# Autodesk Inventor assembly: Internal Wide Panels
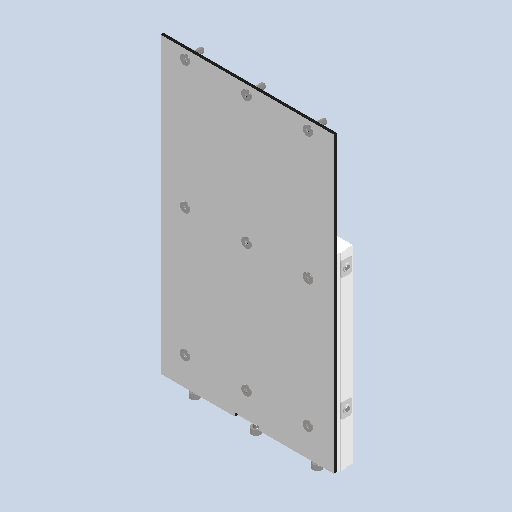
[picture p0: Inventor's stored thumbnail of the model, 512x512]
Saved by Autodesk Inventor 2024 (Build 280153000, 153)
## iProperties
Created: 2024-09-28
Part Number: Internal Wide Panels
Document SubType Name: Assembly
Designer: Ishaan
Author: Ishaan
## Documents named in this file (8)
- E:\Projects\Axiom--IDEX-3D-Printer\CAD\08 - Side Panelling\Internal Wide Panels.iam
- E:\Projects\Axiom--IDEX-3D-Printer\CAD\08 - Side Panelling\Internal medium panel supports.ipt
- E:\Projects\Axiom--IDEX-3D-Printer\CAD\08 - Side Panelling\Medium Internal Vertical Side Panels.ipt
- E:\Projects\Axiom--IDEX-3D-Printer\CAD\00 - COTS Components\Hardware\SHCSM5x12.ipt
- E:\Projects\Axiom--IDEX-3D-Printer\CAD\00 - COTS Components\Hardware\M5 LOCKNUT.ipt
- E:\Projects\Axiom--IDEX-3D-Printer\CAD\00 - COTS Components\Hardware\M5 T SLOT NUT.ipt
- E:\Projects\Axiom--IDEX-3D-Printer\CAD\00 - COTS Components\Hardware\Low Profile M5x16.ipt
- E:\Projects\Axiom--IDEX-3D-Printer\CAD\00 - COTS Components\Hardware\SHCSM5x16.ipt
## Components (31 placed, 7 different names)
1. Internal medium panel supports:1 — Insert:1, Insert:2, Insert:3, Insert:4, Insert:5, Insert:6, Insert:7, Insert:8, Insert:9, Insert:10, Insert:11, Insert:12, Insert:13, Insert:14, Insert:15, Insert:16, Insert:17, Insert:18, Insert:19, Angle:1, Angle:2, Angle:3, Angle:4, Angle:5, Angle:6, Angle:7, Angle:8, Angle:9, Insert:20, Insert:21, Insert:22, Insert:23, Angle:10, Angle:11, Angle:12, Angle:13, Insert:33, Insert:34, Insert:35
2. Medium Internal Vertical Side Panels:1 — Insert:1, Insert:2, Insert:3, Insert:4, Insert:5, Insert:6, Insert:24, Insert:25, Insert:26, Insert:27, Insert:28, Insert:29, Insert:30, Insert:31, Insert:32
3. SHCSM5x12:1 — Insert:10
4. SHCSM5x12:2 — Insert:9
5. SHCSM5x12:3 — Insert:8
6. SHCSM5x12:4 — Insert:7
7. M5 LOCKNUT:1 — Insert:17, Angle:3
8. M5 LOCKNUT:2 — Insert:15, Angle:8
9. M5 LOCKNUT:3 — Insert:18, Angle:2
10. M5 LOCKNUT:4 — Insert:19, Angle:1
11. M5 LOCKNUT:5 — Insert:16, Angle:9
12. M5 LOCKNUT:6 — Insert:14, Angle:7
13. M5 LOCKNUT:7 — Insert:11, Angle:6
14. M5 LOCKNUT:8 — Insert:12, Angle:5
15. M5 LOCKNUT:9 — Insert:13, Angle:4
16. M5 T SLOT NUT:1 — Insert:23, Angle:10
17. M5 T SLOT NUT:2 — Insert:22, Angle:11
18. M5 T SLOT NUT:3 — Insert:21, Angle:13
19. M5 T SLOT NUT:4 — Insert:20, Angle:12
20. Low Profile M5x16:1 — Insert:24
21. Low Profile M5x16:5 — Insert:32
22. Low Profile M5x16:6 — Insert:25
23. Low Profile M5x16:7 — Insert:26
24. Low Profile M5x16:8 — Insert:30
25. Low Profile M5x16:9 — Insert:31
26. Low Profile M5x16:10 — Insert:29
27. Low Profile M5x16:11 — Insert:28
28. Low Profile M5x16:12 — Insert:27
29. SHCSM5x16:1 — Insert:33
30. SHCSM5x16:2 — Insert:35
31. SHCSM5x16:3 — Insert:34
## Relationships (48: Insert 35, Angle 13)
- Insert:1: Internal medium panel supports:1 ↔ Medium Internal Vertical Side Panels:1
- Insert:2: Internal medium panel supports:1 ↔ Medium Internal Vertical Side Panels:1
- Insert:3: Internal medium panel supports:1 ↔ Medium Internal Vertical Side Panels:1
- Insert:4: Internal medium panel supports:1 ↔ Medium Internal Vertical Side Panels:1
- Insert:5: Internal medium panel supports:1 ↔ Medium Internal Vertical Side Panels:1
- Insert:6: Internal medium panel supports:1 ↔ Medium Internal Vertical Side Panels:1
- Insert:7: Internal medium panel supports:1 ↔ SHCSM5x12:4
- Insert:8: Internal medium panel supports:1 ↔ SHCSM5x12:3
- Insert:9: Internal medium panel supports:1 ↔ SHCSM5x12:2
- Insert:10: Internal medium panel supports:1 ↔ SHCSM5x12:1
- Insert:11: Internal medium panel supports:1 ↔ M5 LOCKNUT:7
- Insert:12: Internal medium panel supports:1 ↔ M5 LOCKNUT:8
- Insert:13: Internal medium panel supports:1 ↔ M5 LOCKNUT:9
- Insert:14: Internal medium panel supports:1 ↔ M5 LOCKNUT:6
- Insert:15: Internal medium panel supports:1 ↔ M5 LOCKNUT:2
- Insert:16: Internal medium panel supports:1 ↔ M5 LOCKNUT:5
- Insert:17: Internal medium panel supports:1 ↔ M5 LOCKNUT:1
- Insert:18: Internal medium panel supports:1 ↔ M5 LOCKNUT:3
- Insert:19: Internal medium panel supports:1 ↔ M5 LOCKNUT:4
- Angle:1 (0 deg): Internal medium panel supports:1 ↔ M5 LOCKNUT:4
- Angle:2 (0 deg): Internal medium panel supports:1 ↔ M5 LOCKNUT:3
- Angle:3 (0 deg): Internal medium panel supports:1 ↔ M5 LOCKNUT:1
- Angle:4 (0 deg): Internal medium panel supports:1 ↔ M5 LOCKNUT:9
- Angle:5 (0 deg): Internal medium panel supports:1 ↔ M5 LOCKNUT:8
- Angle:6 (0 deg): Internal medium panel supports:1 ↔ M5 LOCKNUT:7
- Angle:7 (0 deg): Internal medium panel supports:1 ↔ M5 LOCKNUT:6
- Angle:8 (0 deg): Internal medium panel supports:1 ↔ M5 LOCKNUT:2
- Angle:9 (0 deg): Internal medium panel supports:1 ↔ M5 LOCKNUT:5
- Insert:20 (2 mm): Internal medium panel supports:1 ↔ M5 T SLOT NUT:4
- Insert:21 (2 mm): Internal medium panel supports:1 ↔ M5 T SLOT NUT:3
- Insert:22 (2 mm): Internal medium panel supports:1 ↔ M5 T SLOT NUT:2
- Insert:23 (2 mm): Internal medium panel supports:1 ↔ M5 T SLOT NUT:1
- Angle:10 (0 deg): Internal medium panel supports:1 ↔ M5 T SLOT NUT:1
- Angle:11 (0 deg): Internal medium panel supports:1 ↔ M5 T SLOT NUT:2
- Angle:12 (0 deg): Internal medium panel supports:1 ↔ M5 T SLOT NUT:4
- Angle:13 (0 deg): Internal medium panel supports:1 ↔ M5 T SLOT NUT:3
- Insert:24: Medium Internal Vertical Side Panels:1 ↔ Low Profile M5x16:1
- Insert:25: Medium Internal Vertical Side Panels:1 ↔ Low Profile M5x16:6
- Insert:26: Medium Internal Vertical Side Panels:1 ↔ Low Profile M5x16:7
- Insert:27: Medium Internal Vertical Side Panels:1 ↔ Low Profile M5x16:12
- Insert:28: Medium Internal Vertical Side Panels:1 ↔ Low Profile M5x16:11
- Insert:29: Medium Internal Vertical Side Panels:1 ↔ Low Profile M5x16:10
- Insert:30: Medium Internal Vertical Side Panels:1 ↔ Low Profile M5x16:8
- Insert:31: Medium Internal Vertical Side Panels:1 ↔ Low Profile M5x16:9
- Insert:32: Medium Internal Vertical Side Panels:1 ↔ Low Profile M5x16:5
- Insert:33 (6.35 mm): Internal medium panel supports:1 ↔ SHCSM5x16:1
- Insert:34 (6.35 mm): Internal medium panel supports:1 ↔ SHCSM5x16:3
- Insert:35 (6.35 mm): Internal medium panel supports:1 ↔ SHCSM5x16:2
